# Autodesk Inventor assembly: Center Assembly
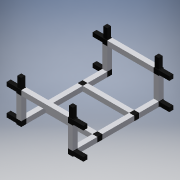
[picture p0: Inventor's stored thumbnail of the model, 180x180]
Saved by Autodesk Inventor 2017 (Build 210142000, 142)
## iProperties
Created: 2019-12-06
Part Number: Center Assembly
Document SubType Name: Assembly
Designer: S346553810
Author: S346553810
## Documents named in this file (2)
- \\ad.ocdsb.ca\studenthome\3\S338674153\FRC 2020\FullRobotRefactor\SubFrame\Center Assembly.iam
- \\ad.ocdsb.ca\studenthome\3\S338674153\FRC 2020\FullRobotRefactor\SubFrame\center cross-member.iam
## Components (2 placed, 1 different names)
1. center cross-member:1 [sub-assembly] — Flush:1, Flush:2, Mate:1
2. center cross-member:2 [sub-assembly] — Flush:1, Flush:2, Mate:1
## Relationships (3: Flush 2, Mate 1)
- Flush:1: center cross-member:1 ↔ center cross-member:2
- Flush:2: center cross-member:1 ↔ center cross-member:2
- Mate:1: center cross-member:1 ↔ center cross-member:2
